# Autodesk Inventor assembly: 090 ASY bottom
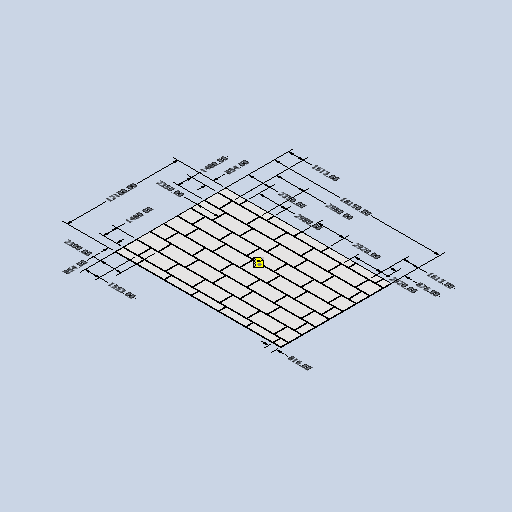
[picture p0: Inventor's stored thumbnail of the model, 512x512]
Saved by Autodesk Inventor 2026.2 (Build 302298010, 298A)
## iProperties
Created: 2026-05-19
Part Number: 090 ASY bottom
Document SubType Name: Assembly
Designer: user
Mass: 1.0309e+07 g
Surface Area: 5.30613e+06 cm^2
Volume: 1.31325e+06 cm^3
Density: 7.85 g/cm^3
Stock Number: 0100
Author: user
## Documents named in this file (8)
- C:\Users\admin\Documents\Inventor\GBK-Gubkinskiy\090 ASY bottom.iam
- C:\Users\admin\Documents\Inventor\GBK-Gubkinskiy\ASY GBK bottom 0010.iam
- C:\Users\admin\Documents\Inventor\GBK-Gubkinskiy\ASY GBK bottom 0020.iam
- C:\Users\admin\Documents\Inventor\GBK-Gubkinskiy\ASY GBK bottom 0021.iam
- C:\Users\admin\Documents\Inventor\GBK-Gubkinskiy\ASY GBK bottom 0022.iam
- C:\Users\admin\Documents\Inventor\GBK-Gubkinskiy\ASY GBK bottom 0023.iam
- C:\Users\admin\Documents\Inventor\GBK-Gubkinskiy\ASY GBK bottom 0021_CPY.iam
- C:\Users\admin\Documents\Inventor\GBK-Gubkinskiy\ASY GBK bottom 0024.iam
## Components (63 placed, 7 different names)
1. ASY GBK bottom 0010:3 [sub-assembly] — Rigid:54
2. ASY GBK bottom 0010:2 [sub-assembly] — Rigid:37, Rigid:50
3. ASY GBK bottom 0010:1 [sub-assembly] — Rigid:37
4. ASY GBK bottom 0020:1 [sub-assembly] — Rigid:45
5. ASY GBK bottom 0020:2 [sub-assembly] — Rigid:45, Rigid:46
6. ASY GBK bottom 0020:3 [sub-assembly] — Rigid:46, Rigid:48
7. ASY GBK bottom 0020:4 [sub-assembly] — Rigid:48, Rigid:49
8. ASY GBK bottom 0020:5 [sub-assembly] — Rigid:49, Rigid:94
9. ASY GBK bottom 0021:1 [sub-assembly] — Rigid:94
10. ASY GBK bottom 0022:1 [sub-assembly] — Flush:3
11. ASY GBK bottom 0023:1 [sub-assembly]
12. ASY GBK bottom 0010:4 [sub-assembly] — Rigid:50, Rigid:51
13. ASY GBK bottom 0010:5 [sub-assembly] — Rigid:51, Rigid:52
14. ASY GBK bottom 0010:6 [sub-assembly] — Rigid:52, Rigid:53
15. ASY GBK bottom 0023:2 [sub-assembly] — Rigid:53
16. ASY GBK bottom 0010:7 [sub-assembly] — Rigid:54, Rigid:55
17. ASY GBK bottom 0010:8 [sub-assembly] — Rigid:55, Rigid:56
18. ASY GBK bottom 0010:9 [sub-assembly] — Rigid:56, Rigid:57
19. ASY GBK bottom 0010:10 [sub-assembly] — Rigid:57, Rigid:58
20. ASY GBK bottom 0025:1 [sub-assembly] — Rigid:58
21. ASY GBK bottom 0010:11 [sub-assembly]
22. ASY GBK bottom 0010:12 [sub-assembly]
23. ASY GBK bottom 0023:3 [sub-assembly] — Rigid:72
24. ASY GBK bottom 0010:13 [sub-assembly]
25. ASY GBK bottom 0010:14 [sub-assembly]
26. ASY GBK bottom 0010:15 [sub-assembly]
27. ASY GBK bottom 0023:4 [sub-assembly]
28. ASY GBK bottom 0024:1 [sub-assembly]
29. ASY GBK bottom 0010:16 [sub-assembly]
30. ASY GBK bottom 0010:17 [sub-assembly]
31. ASY GBK bottom 0010:18 [sub-assembly]
32. ASY GBK bottom 0010:19 [sub-assembly]
33. ASY GBK bottom 0010:20 [sub-assembly]
34. ASY GBK bottom 0025:2 [sub-assembly]
35. ASY GBK bottom 0024:2 [sub-assembly] — Rigid:72, Rigid:79
36. ASY GBK bottom 0010:21 [sub-assembly]
37. ASY GBK bottom 0010:22 [sub-assembly]
38. ASY GBK bottom 0023:5 [sub-assembly] — Rigid:79, Rigid:86
39. ASY GBK bottom 0010:23 [sub-assembly]
40. ASY GBK bottom 0010:24 [sub-assembly]
41. ASY GBK bottom 0010:25 [sub-assembly]
42. ASY GBK bottom 0023:6 [sub-assembly]
43. ASY GBK bottom 0010:26 [sub-assembly]
44. ASY GBK bottom 0010:27 [sub-assembly]
45. ASY GBK bottom 0010:28 [sub-assembly]
46. ASY GBK bottom 0010:29 [sub-assembly]
47. ASY GBK bottom 0010:30 [sub-assembly]
48. ASY GBK bottom 0025:3 [sub-assembly]
49. ASY GBK bottom 0024:3 [sub-assembly] — Rigid:86, Rigid:93
50. ASY GBK bottom 0010:31 [sub-assembly]
51. ASY GBK bottom 0010:32 [sub-assembly]
52. ASY GBK bottom 0023:7 [sub-assembly] — Rigid:93, Rigid:101
53. ASY GBK bottom 0010:33 [sub-assembly]
54. ASY GBK bottom 0010:34 [sub-assembly]
55. ASY GBK bottom 0010:35 [sub-assembly]
56. ASY GBK bottom 0023:8 [sub-assembly]
57. ASY GBK bottom 0020:6 [sub-assembly]
58. ASY GBK bottom 0020:7 [sub-assembly]
59. ASY GBK bottom 0020:8 [sub-assembly]
60. ASY GBK bottom 0020:9 [sub-assembly]
61. ASY GBK bottom 0020:10 [sub-assembly]
62. ASY GBK bottom 0021:2 [sub-assembly]
63. ASY GBK bottom 0022:2 [sub-assembly] — Rigid:101
## Relationships (65: WeldJoint 62, Mate 2, Flush 1)
- [WeldJoint] (4 mm): ASY GBK bottom 0010:1 ↔ ASY GBK bottom 0023:1
- [Mate] (-9075 mm): ASY GBK bottom 0023:1
- [WeldJoint] (4 mm): ASY GBK bottom 0022:1 ↔ ASY GBK bottom 0023:1
- Flush:3: ASY GBK bottom 0022:1
- [Mate] (-6050 mm): ASY GBK bottom 0022:1
- [WeldJoint] (4 mm): ASY GBK bottom 0020:1 ↔ ASY GBK bottom 0022:1
- [WeldJoint] (4 mm): ASY GBK bottom 0023:1 ↔ ASY GBK bottom 0024:1
- Rigid:37 [WeldJoint] (4 mm): ASY GBK bottom 0010:2 ↔ ASY GBK bottom 0010:1
- [WeldJoint] (4 mm): ASY GBK bottom 0010:3 ↔ ASY GBK bottom 0024:1
- Rigid:45 [WeldJoint] (4 mm): ASY GBK bottom 0020:1 ↔ ASY GBK bottom 0020:2
- Rigid:46 [WeldJoint] (4 mm): ASY GBK bottom 0020:2 ↔ ASY GBK bottom 0020:3
- Rigid:48 [WeldJoint] (4 mm): ASY GBK bottom 0020:3 ↔ ASY GBK bottom 0020:4
- Rigid:49 [WeldJoint] (4 mm): ASY GBK bottom 0020:4 ↔ ASY GBK bottom 0020:5
- Rigid:50 [WeldJoint] (4 mm): ASY GBK bottom 0010:2 ↔ ASY GBK bottom 0010:4
- Rigid:51 [WeldJoint] (4 mm): ASY GBK bottom 0010:4 ↔ ASY GBK bottom 0010:5
- Rigid:52 [WeldJoint] (4 mm): ASY GBK bottom 0010:5 ↔ ASY GBK bottom 0010:6
- Rigid:53 [WeldJoint] (4 mm): ASY GBK bottom 0010:6 ↔ ASY GBK bottom 0023:2
- Rigid:54 [WeldJoint] (4 mm): ASY GBK bottom 0010:3 ↔ ASY GBK bottom 0010:7
- Rigid:55 [WeldJoint] (4 mm): ASY GBK bottom 0010:7 ↔ ASY GBK bottom 0010:8
- Rigid:56 [WeldJoint] (4 mm): ASY GBK bottom 0010:8 ↔ ASY GBK bottom 0010:9
- Rigid:57 [WeldJoint] (4 mm): ASY GBK bottom 0010:9 ↔ ASY GBK bottom 0010:10
- Rigid:58 [WeldJoint] (4 mm): ASY GBK bottom 0010:10 ↔ ASY GBK bottom 0025:1
- [WeldJoint] (4 mm): ASY GBK bottom 0010:11 ↔ ASY GBK bottom 0023:3
- [WeldJoint] (4 mm): ASY GBK bottom 0010:11 ↔ ASY GBK bottom 0010:12
- [WeldJoint] (4 mm): ASY GBK bottom 0010:12 ↔ ASY GBK bottom 0010:13
- [WeldJoint] (4 mm): ASY GBK bottom 0010:13 ↔ ASY GBK bottom 0010:14
- [WeldJoint] (4 mm): ASY GBK bottom 0010:14 ↔ ASY GBK bottom 0010:15
- [WeldJoint] (4 mm): ASY GBK bottom 0010:15 ↔ ASY GBK bottom 0023:4
- [WeldJoint] (4 mm): ASY GBK bottom 0023:3 ↔ ASY GBK bottom 0024:1
- [WeldJoint] (4 mm): ASY GBK bottom 0010:16 ↔ ASY GBK bottom 0024:2
- [WeldJoint] (4 mm): ASY GBK bottom 0010:16 ↔ ASY GBK bottom 0010:17
- [WeldJoint] (4 mm): ASY GBK bottom 0010:17 ↔ ASY GBK bottom 0010:18
- [WeldJoint] (4 mm): ASY GBK bottom 0010:18 ↔ ASY GBK bottom 0010:19
- [WeldJoint] (4 mm): ASY GBK bottom 0010:19 ↔ ASY GBK bottom 0010:20
- [WeldJoint] (4 mm): ASY GBK bottom 0010:20 ↔ ASY GBK bottom 0025:2
- Rigid:72 [WeldJoint] (4 mm): ASY GBK bottom 0023:3 ↔ ASY GBK bottom 0024:2
- [WeldJoint] (4 mm): ASY GBK bottom 0010:21 ↔ ASY GBK bottom 0023:5
- [WeldJoint] (4 mm): ASY GBK bottom 0010:21 ↔ ASY GBK bottom 0010:22
- [WeldJoint] (4 mm): ASY GBK bottom 0010:22 ↔ ASY GBK bottom 0010:23
- [WeldJoint] (4 mm): ASY GBK bottom 0010:23 ↔ ASY GBK bottom 0010:24
- [WeldJoint] (4 mm): ASY GBK bottom 0010:24 ↔ ASY GBK bottom 0010:25
- [WeldJoint] (4 mm): ASY GBK bottom 0010:25 ↔ ASY GBK bottom 0023:6
- Rigid:79 [WeldJoint] (4 mm): ASY GBK bottom 0024:2 ↔ ASY GBK bottom 0023:5
- [WeldJoint] (4 mm): ASY GBK bottom 0010:26 ↔ ASY GBK bottom 0024:3
- [WeldJoint] (4 mm): ASY GBK bottom 0010:26 ↔ ASY GBK bottom 0010:27
- [WeldJoint] (4 mm): ASY GBK bottom 0010:27 ↔ ASY GBK bottom 0010:28
- [WeldJoint] (4 mm): ASY GBK bottom 0010:28 ↔ ASY GBK bottom 0010:29
- [WeldJoint] (4 mm): ASY GBK bottom 0010:29 ↔ ASY GBK bottom 0010:30
- [WeldJoint] (4 mm): ASY GBK bottom 0010:30 ↔ ASY GBK bottom 0025:3
- Rigid:86 [WeldJoint] (4 mm): ASY GBK bottom 0023:5 ↔ ASY GBK bottom 0024:3
- [WeldJoint] (4 mm): ASY GBK bottom 0010:31 ↔ ASY GBK bottom 0023:7
- [WeldJoint] (4 mm): ASY GBK bottom 0010:31 ↔ ASY GBK bottom 0010:32
- [WeldJoint] (4 mm): ASY GBK bottom 0010:32 ↔ ASY GBK bottom 0010:33
- [WeldJoint] (4 mm): ASY GBK bottom 0010:33 ↔ ASY GBK bottom 0010:34
- [WeldJoint] (4 mm): ASY GBK bottom 0010:34 ↔ ASY GBK bottom 0010:35
- [WeldJoint] (4 mm): ASY GBK bottom 0010:35 ↔ ASY GBK bottom 0023:8
- Rigid:93 [WeldJoint] (4 mm): ASY GBK bottom 0024:3 ↔ ASY GBK bottom 0023:7
- Rigid:94 [WeldJoint] (4 mm): ASY GBK bottom 0020:5 ↔ ASY GBK bottom 0021:1
- [WeldJoint] (4 mm): ASY GBK bottom 0020:6 ↔ ASY GBK bottom 0022:2
- [WeldJoint] (4 mm): ASY GBK bottom 0020:6 ↔ ASY GBK bottom 0020:7
- [WeldJoint] (4 mm): ASY GBK bottom 0020:7 ↔ ASY GBK bottom 0020:8
- [WeldJoint] (4 mm): ASY GBK bottom 0020:8 ↔ ASY GBK bottom 0020:9
- [WeldJoint] (4 mm): ASY GBK bottom 0020:9 ↔ ASY GBK bottom 0020:10
- [WeldJoint] (4 mm): ASY GBK bottom 0020:10 ↔ ASY GBK bottom 0021:2
- Rigid:101 [WeldJoint] (4 mm): ASY GBK bottom 0023:7 ↔ ASY GBK bottom 0022:2
## Named parameters: d154_d147 = 4 mm, d155_d148 = 4 mm, d156_d111 = 4 mm, d157_d145 = 4 mm, d158_d146 = 4 mm, d159_d37 = 4 mm, d161_d149 = 4 mm, d162_d150 = 4 mm, d163_d151 = 4 mm, d164_d152 = 4 mm, d165_d153 = 4 mm, d166_d113 = 4 mm, d168_d147 = 4 mm, d169_d148 = 4 mm, d170_d111 = 4 mm, d171_d145 = 4 mm, d172_d146 = 4 mm, d173_d37 = 4 mm, d175_d149 = 4 mm, d176_d150 = 4 mm, d177_d151 = 4 mm, d178_d152 = 4 mm, d179_d153 = 4 mm, d180_d113 = 4 mm, d188_d147 = 4 mm, d189_d148 = 4 mm, d190_d111 = 4 mm, d191_d145 = 4 mm, d192_d146 = 4 mm, d193_d37 = 4 mm, d196_d195 = 4 mm, d197_d137 = 4 mm, d198_d138 = 4 mm, d199_d140 = 4 mm, d200_d141 = 4 mm, d201_d76 = 4 mm
